# Autodesk Inventor assembly: blocmoteur
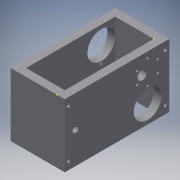
[picture p0: Inventor's stored thumbnail of the model, 180x180]
Saved by Autodesk Inventor 2017 SP1 (Build 210196100, 196)
## iProperties
Part Number: blocmoteur
Material: Générique
Document SubType Name: Assembly
Designer: Sylvain
Author: Sylvain
## Documents named in this file (3)
- C:\Users\Sylvain\Desktop\PetitRobot3D\blocmoteur.iam
- C:\Users\Sylvain\Desktop\PetitRobot3D\paroismoteur.ipt
- C:\Users\Sylvain\Desktop\PetitRobot3D\spacermoteur.ipt
## Components (4 placed, 2 different names)
1. paroismoteur:1 — Placage:8, Placage:9
2. paroismoteur:2 — Placage:1, Placage:3, Placage:5, Placage:7, Placage:10, Placage:11
3. spacermoteur:1 — Placage:3, Placage:7
4. spacermoteur:2 — Placage:1, Placage:5, Placage:8, Placage:9, Placage:10, Placage:11
## Relationships (8: Mate 8)
- Placage:1 [Mate]: paroismoteur:2 ↔ spacermoteur:2
- Placage:3 [Mate]: paroismoteur:2 ↔ spacermoteur:1
- Placage:5 [Mate]: paroismoteur:2 ↔ spacermoteur:2
- Placage:7 [Mate]: paroismoteur:2 ↔ spacermoteur:1
- Placage:8 [Mate]: paroismoteur:1 ↔ spacermoteur:2
- Placage:9 [Mate]: paroismoteur:1 ↔ spacermoteur:2
- Placage:10 [Mate]: paroismoteur:2 ↔ spacermoteur:2
- Placage:11 [Mate]: paroismoteur:2 ↔ spacermoteur:2
